# Autodesk Inventor assembly: Plasma-box-hayashi-aka-upgrade
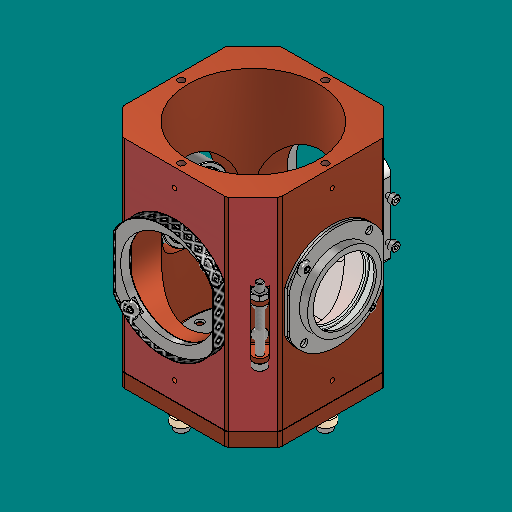
[picture p0: Inventor's stored thumbnail of the model, 512x512]
Saved by Autodesk Inventor 2025 (Build 290162000, 162)
## iProperties
Created: 2024-05-15
Part Number: Plasma-box-hayashi-aka-upgrade
Document SubType Name: Assembly
Designer: kuzmin
Mass: 1430.79 g
Surface Area: 719.778 cm^2
Volume: 163.414 cm^3
Density: 8.75564 g/cm^3
Author: kuzmin
## iProperties of the stored document MemberDocs/xCzzmitmsH0puyzanWmilobey5h
Created: 2024-05-15
Part Number: Plasma-box-hayashi-aka-upgrade
Document SubType Name: Assembly
Designer: kuzmin
Mass: 1430.79 g
Surface Area: 719.778 cm^2
Volume: 163.414 cm^3
Density: 8.75564 g/cm^3
Author: kuzmin
## Documents named in this file (17)
- C:\Users\queez\Dropbox\Drawings\PIHTI\Plasma Vessel\Plasma-Box\Plasma-box-for-boron.iam
- C:\Users\queez\Dropbox\Drawings\PIHTI\Plasma Vessel\Plasma-Box\plasma_box.ipt
- C:\Users\queez\Dropbox\Drawings\PIHTI\Plasma Vessel\Plasma-Box\plasma-box-hinge.ipt
- C:\Users\queez\Dropbox\Drawings\PIHTI\ContentCenter\Fastners\M3x8-BHCS.ipt
- C:\Users\queez\Dropbox\Drawings\PIHTI\ContentCenter\Fastners\M3x30-SHCS.ipt
- C:\Users\queez\Dropbox\Drawings\PIHTI\ContentCenter\Fastners\M3-nut.ipt
- C:\Users\queez\Dropbox\Drawings\PIHTI\Plasma Vessel\Plasma-Box\probe-gate-spacer.ipt
- C:\Users\queez\Dropbox\Drawings\PIHTI\Plasma Vessel\Plasma-Box\probe-gate-mesh.ipt
- C:\Users\queez\Dropbox\Drawings\PIHTI\Plasma Vessel\Plasma-Box\plasma-box-slit-to-cathode.ipt
- C:\Users\queez\Dropbox\Drawings\PIHTI\Plasma Vessel\Plasma-Box\probe-gate-spacer\probe-gate-spacer-angled.ipt
- C:\Users\queez\Dropbox\Drawings\PIHTI\Plasma Vessel\Plasma-Box\quartz-window-30mm-in-holder.iam
- C:\Users\queez\Dropbox\Drawings\PIHTI\Plasma Vessel\Plasma-Box\probe-gate-spacer\probe-gate-spacer-40mm-mesh-holder.ipt
- C:\Users\queez\Dropbox\Drawings\PIHTI\ContentCenter\Fastners\M2x4-SHCS.ipt
- C:\Users\queez\Dropbox\Drawings\PIHTI\Plasma Vessel\Plasma-Box\probe-gate-with-spindel.iam
- C:\Users\queez\Dropbox\Drawings\PIHTI\Plasma Vessel\Plasma-Box\plasma-box-to-cathode-box-adapter.iam
- C:\Users\queez\Dropbox\Drawings\PIHTI\Plasma Vessel\Boron-Target\boron-dish.ipt
- C:\Users\queez\Dropbox\Drawings\PIHTI\Plasma Vessel\Plasma-Box\mesh-window-35mm-assembly.iam
## Components (24 placed, 15 different names)
1. plasma_box:1 — Flush:1, Flush:2, Flush:3, Mate:1, Mate:2, Mate:3, Mate:4, Mate:5, Mate:7, Mate:8, Rigid:12, Rotational:5, Rigid:15, Rigid:16, Rotational:6, Rigid:17, Rigid:18, Mate:14, Mate:15, Mate:16, Mate:17, Mate:18, Rigid:19, Rigid:20, Mate:26, Mate:27
2. plasma-box-hinge:1 — Mate:1, Mate:2, Mate:3, Rotational:1, Rigid:7, Rotational:2, Rotational:3, Mate:19, Mate:20
3. probe-gate-spacer-angled:1 — Mate:4, Mate:5, Angle:1, Mate:16
4. probe-gate-mesh:1 — Mate:7, Mate:8, Angle:1
5. plasma-box-slit-to-cathode:1
6. quartz-window-30mm-in-holder:1 [sub-assembly] — Rotational:6, Mate:17
7. probe-gate-spacer-40mm-mesh-holder:2 — Mate:14, Mate:15, Mate:18, Rigid:23
8. probe-gate-with-spindel:1 [sub-assembly] — Mate:19, Mate:20
9. plasma-box-to-cathode-box-adapter:1 [sub-assembly] — Mate:26
10. boron-dish:1 — Mate:27
11. SS ISO 4762 M2 x 4:1
12. SS ISO 4762 M2 x 4:2 — Rigid:23
13. BS 4168 : Part 6 Hexagon socket countersunk and button head screws - Metric series - Metric M3 x 8:10 — Rigid:20
14. BS 4168 : Part 6 Hexagon socket countersunk and button head screws - Metric series - Metric M3 x 8:9 — Rigid:19
15. BS 4168 : Part 6 Hexagon socket countersunk and button head screws - Metric series - Metric M3 x 8:7 — Rigid:17
16. BS 4168 : Part 6 Hexagon socket countersunk and button head screws - Metric series - Metric M3 x 8:8 — Rigid:18
17. M3x8-BHSC:1 — Rigid:15
18. M3x8-BHSC:2 — Rigid:16
19. M3x8-BHSC:3 — Rigid:12
20. M3x8-BHSC:4 — Rotational:5
21. M3x8-BHSC:5 — Rotational:1
22. M3x8-BHSC:6 — Rigid:7
23. UNI 5931 M 3 x  30:1 — Rotational:2
24. JIS B 1181 Style 1 - Metric A M3:1 — Rotational:3
## Relationships (36: Mate 18, WeldJoint 9, RevoluteJoint 5, Flush 3, Angle 1)
- Flush:1: plasma_box:1
- Flush:2: plasma_box:1
- Flush:3: plasma_box:1
- Mate:1: plasma_box:1 ↔ plasma-box-hinge:1
- Mate:2: plasma_box:1 ↔ plasma-box-hinge:1
- Mate:3: plasma_box:1 ↔ plasma-box-hinge:1
- Rotational:1 [RevoluteJoint]: plasma-box-hinge:1 ↔ M3x8-BHSC:5
- Rigid:7 [WeldJoint]: plasma-box-hinge:1 ↔ M3x8-BHSC:6
- Rotational:2 [RevoluteJoint]: plasma-box-hinge:1 ↔ UNI 5931 M 3 x  30:1
- Rotational:3 [RevoluteJoint]: plasma-box-hinge:1 ↔ JIS B 1181 Style 1 - Metric A M3:1
- Mate:4 (0.2 mm): plasma_box:1 ↔ probe-gate-spacer-angled:1
- Mate:5: plasma_box:1 ↔ probe-gate-spacer-angled:1
- Mate:7: plasma_box:1 ↔ probe-gate-mesh:1
- Mate:8: plasma_box:1 ↔ probe-gate-mesh:1
- Angle:1 (0 deg): probe-gate-spacer-angled:1 ↔ probe-gate-mesh:1
- Rigid:12 [WeldJoint] (1.7 mm): plasma_box:1 ↔ M3x8-BHSC:3
- Rotational:5 [RevoluteJoint] (1.7 mm): plasma_box:1 ↔ M3x8-BHSC:4
- Rigid:15 [WeldJoint] (-1.7 mm): plasma_box:1 ↔ M3x8-BHSC:1
- Rigid:16 [WeldJoint] (-1.7 mm): plasma_box:1 ↔ M3x8-BHSC:2
- Rotational:6 [RevoluteJoint]: plasma_box:1 ↔ quartz-window-30mm-in-holder:1
- Rigid:17 [WeldJoint] (1.7 mm): plasma_box:1 ↔ BS 4168 : Part 6 Hexagon socket countersunk and button head screws - Metric series - Metric M3 x 8:7
- Rigid:18 [WeldJoint] (1.7 mm): plasma_box:1 ↔ BS 4168 : Part 6 Hexagon socket countersunk and button head screws - Metric series - Metric M3 x 8:8
- Mate:14: plasma_box:1 ↔ probe-gate-spacer-40mm-mesh-holder:2
- Mate:15: plasma_box:1 ↔ probe-gate-spacer-40mm-mesh-holder:2
- Mate:16: plasma_box:1 ↔ probe-gate-spacer-angled:1
- Mate:17: plasma_box:1 ↔ quartz-window-30mm-in-holder:1
- Mate:18: plasma_box:1 ↔ probe-gate-spacer-40mm-mesh-holder:2
- Rigid:19 [WeldJoint] (1.5 mm): plasma_box:1 ↔ BS 4168 : Part 6 Hexagon socket countersunk and button head screws - Metric series - Metric M3 x 8:9
- Rigid:20 [WeldJoint] (1.5 mm): plasma_box:1 ↔ BS 4168 : Part 6 Hexagon socket countersunk and button head screws - Metric series - Metric M3 x 8:10
- Rigid:23 [WeldJoint] (-2 mm): probe-gate-spacer-40mm-mesh-holder:2 ↔ SS ISO 4762 M2 x 4:2
- Mate:19: plasma-box-hinge:1 ↔ probe-gate-with-spindel:1
- Mate:20: plasma-box-hinge:1 ↔ probe-gate-with-spindel:1
- [Mate]: plasma_box:1 ↔ plasma-box-to-cathode-box-adapter:1
- [Mate]: plasma_box:1 ↔ plasma-box-to-cathode-box-adapter:1
- Mate:26: plasma_box:1 ↔ plasma-box-to-cathode-box-adapter:1
- Mate:27: plasma_box:1 ↔ boron-dish:1
